# Autodesk Inventor assembly: MIR_HbthumbU02ForChild1
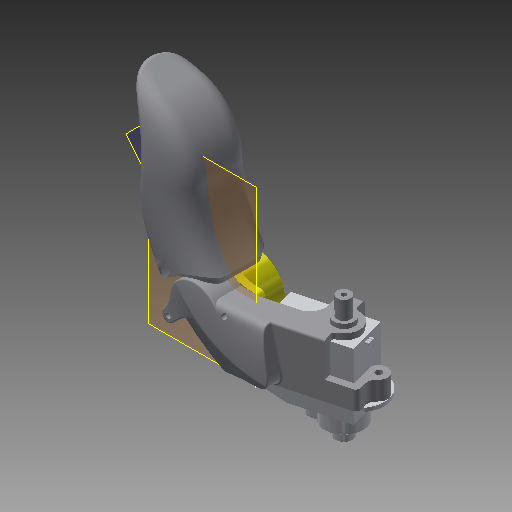
[picture p0: Inventor's stored thumbnail of the model, 512x512]
Saved by Autodesk Inventor 2018.1 (Build 221171000, 171)
## iProperties
Part Number: MIR_HbthumbU02ForChild1
Material: 一般
Document SubType Name: Assembly
Designer: sktom
Author: sktom
## Documents named in this file (8)
- D:\CloudStrage\OneDrive\CAD\MAJ\hackberry\HACKberry-hardware\3D_69%inlength\Inventor\HbHandForChild\HbthumbU02ForChild\MIR_HbthumbU02ForChild1.iam
- D:\CloudStrage\OneDrive\CAD\MAJ\hackberry\HACKberry-hardware\3D_69%inlength\Inventor\HbHandForChild\HbthumbU02ForChild\MIR_HbThumbMetacarpalPhalanx02ForChild1.ipt
- D:\CloudStrage\OneDrive\CAD\MAJ\hackberry\HACKberry-hardware\3D_69%inlength\Inventor\HbHandForChild\HbthumbU02ForChild\MIR_HbThumbLockButton01ForChild1.ipt
- D:\CloudStrage\OneDrive\CAD\MAJ\hackberry\HACKberry-hardware\3D_69%inlength\Inventor\HbHandForChild\HbthumbU02ForChild\MIR_HbThumbJointHolder01ForChild1.ipt
- D:\CloudStrage\OneDrive\CAD\MAJ\hackberry\HACKberry-hardware\3D_69%inlength\Inventor\HbHandForChild\HbthumbU02ForChild\MIR_HbThumbProximalPhalanx02ForChild1.ipt
- D:\CloudStrage\OneDrive\CAD\MAJ\hackberry\HACKberry-hardware\3D_69%inlength\Inventor\HbHandForChild\HbthumbU02ForChild\MIR_HbThumbProximalPhalanxBase02ForChild1.ipt
- D:\CloudStrage\OneDrive\CAD\MAJ\hackberry\HACKberry-hardware\3D_69%inlength\Inventor\HbHandForChild\HbthumbU02ForChild\MIR_HbThumbMetacarpalPhalanxCover02ForChild1.ipt
- D:\CloudStrage\OneDrive\CAD\MAJ\hackberry\HACKberry-hardware\3D_69%inlength\Inventor\HbHandForChild\HbthumbU02ForChild\HbServoHK282A\MIR_Servo_HK282A1.ipt
## Components (7 placed, 7 different names)
1. MIR_HbThumbMetacarpalPhalanx02ForChild1:1 — 挿入:3, 挿入:2, 挿入:1, 挿入:8, 挿入:7
2. MIR_HbThumbLockButton01ForChild1:1 — 挿入:3
3. MIR_HbThumbJointHolder01ForChild1:1 — 挿入:2, 挿入:1, 挿入:4, 挿入:6
4. MIR_HbThumbProximalPhalanx02ForChild1:1 — 挿入:5
5. MIR_HbThumbProximalPhalanxBase02ForChild1:1 — 挿入:5, 挿入:4
6. MIR_HbThumbMetacarpalPhalanxCover02ForChild1:1 — 挿入:6
7. MIR_Servo_HK282A1:1 — 挿入:8, 挿入:7
## Relationships (8: Insert 8)
- 挿入:3 [Insert] (2 mm): MIR_HbThumbMetacarpalPhalanx02ForChild1:1 ↔ MIR_HbThumbLockButton01ForChild1:1
- 挿入:2 [Insert]: MIR_HbThumbMetacarpalPhalanx02ForChild1:1 ↔ MIR_HbThumbJointHolder01ForChild1:1
- 挿入:1 [Insert]: MIR_HbThumbMetacarpalPhalanx02ForChild1:1 ↔ MIR_HbThumbJointHolder01ForChild1:1
- 挿入:5 [Insert] (0.2 mm): MIR_HbThumbProximalPhalanx02ForChild1:1 ↔ MIR_HbThumbProximalPhalanxBase02ForChild1:1
- 挿入:4 [Insert]: MIR_HbThumbJointHolder01ForChild1:1 ↔ MIR_HbThumbProximalPhalanxBase02ForChild1:1
- 挿入:6 [Insert]: MIR_HbThumbJointHolder01ForChild1:1 ↔ MIR_HbThumbMetacarpalPhalanxCover02ForChild1:1
- 挿入:8 [Insert]: MIR_HbThumbMetacarpalPhalanx02ForChild1:1 ↔ MIR_Servo_HK282A1:1
- 挿入:7 [Insert]: MIR_HbThumbMetacarpalPhalanx02ForChild1:1 ↔ MIR_Servo_HK282A1:1
